# Autodesk Inventor assembly: reducer_1
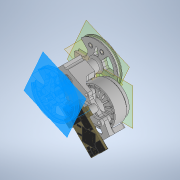
[picture p0: Inventor's stored thumbnail of the model, 180x180]
Saved by Autodesk Inventor 2023 (Build 270158000, 158)
## iProperties
Created: 2020-12-06
Part Number: reducer_1
Document SubType Name: Assembly
Designer: Shuang Peng
Author: Shuang Peng
## Documents named in this file (9)
- D:\projects-3\biped_tiny\hardware\reducer_1.iam
- D:\projects-3\biped_tiny\hardware\mot_27_ass.iam
- D:\projects-3\biped_tiny\hardware\tendon_wh_1.ipt
- D:\projects-3\biped_tiny\hardware\mot_holder_1.ipt
- D:\projects-3\biped_tiny\hardware\bearing_3_6_2.ipt
- D:\projects-3\biped_tiny\hardware\pin_3_15.ipt
- D:\projects-3\biped_tiny\hardware\screw_holder_2_3.ipt
- D:\projects-3\biped_tiny\hardware\encoder_holder_2.ipt
- D:\projects-3\biped_tiny\hardware\eletronic\brushless sub driver 2 v1\brushless sub driver 2.iam
## Components (13 placed, 8 different names)
1. mot_27_ass:1 [sub-assembly] — Flush:1, Insert:1, Insert:2, Flush:2, Insert:3, Insert:4
2. tendon_wh_1:1 — Flush:1, Insert:1, Insert:2, Flush:3
3. mot_holder_1:1 — Flush:2, Insert:3, Insert:4, Insert:5, Insert:14, Insert:15, Insert:16, Flush:4, Insert:18, Insert:19, Insert:28, Insert:29
4. bearing_3_6_2:1 — Insert:5
5. bearing_3_6_2:2 — Insert:8, Insert:16
6. pin_3_15:1 — Insert:8
7. screw_holder_2_3:6 — Insert:14
8. screw_holder_2_3:7 — Insert:15
9. encoder_holder_2:1 — Flush:4, Insert:17, Insert:18, Insert:19, Insert:21
10. screw_holder_2_3:8 — Insert:17, Insert:20
11. brushless sub driver 2:1 [sub-assembly] — Insert:20, Insert:21
12. screw_holder_2_3:14 — Insert:29
13. screw_holder_2_3:15 — Insert:28
## Relationships (20: Insert 16, Flush 4)
- Flush:1: mot_27_ass:1 ↔ tendon_wh_1:1
- Insert:1: mot_27_ass:1 ↔ tendon_wh_1:1
- Insert:2: mot_27_ass:1 ↔ tendon_wh_1:1
- Flush:2: mot_27_ass:1 ↔ mot_holder_1:1
- Insert:3: mot_27_ass:1 ↔ mot_holder_1:1
- Insert:4: mot_27_ass:1 ↔ mot_holder_1:1
- Insert:5: mot_holder_1:1 ↔ bearing_3_6_2:1
- Flush:3 (1.5 mm): tendon_wh_1:1
- Insert:8: bearing_3_6_2:2 ↔ pin_3_15:1
- Insert:14: mot_holder_1:1 ↔ screw_holder_2_3:6
- Insert:15: mot_holder_1:1 ↔ screw_holder_2_3:7
- Insert:16: mot_holder_1:1 ↔ bearing_3_6_2:2
- Flush:4: mot_holder_1:1 ↔ encoder_holder_2:1
- Insert:17: encoder_holder_2:1 ↔ screw_holder_2_3:8
- Insert:18: mot_holder_1:1 ↔ encoder_holder_2:1
- Insert:19: mot_holder_1:1 ↔ encoder_holder_2:1
- Insert:20: screw_holder_2_3:8 ↔ brushless sub driver 2:1
- Insert:21: encoder_holder_2:1 ↔ brushless sub driver 2:1
- Insert:28: mot_holder_1:1 ↔ screw_holder_2_3:15
- Insert:29: mot_holder_1:1 ↔ screw_holder_2_3:14
